# Autodesk Inventor assembly: pinion_assembly
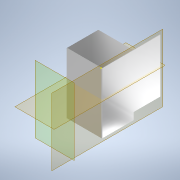
[picture p0: Inventor's stored thumbnail of the model, 180x180]
Saved by Autodesk Inventor 2021 (Build 250183000, 183)
## iProperties
Created: 2021-06-23
Part Number: pinion_assembly
Document SubType Name: Assembly
## Documents named in this file (3)
- C:\Users\ocon0143\OneDrive - Flinders\Advn Mech Design Shared\6_Development\2_Design\inventor\rack_pinion\pinion_assembly.iam
- C:\Users\ocon0143\OneDrive - Flinders\Advn Mech Design Shared\6_Development\2_Design\inventor\support\reel\motor.ipt
- C:\Users\ocon0143\OneDrive - Flinders\Advn Mech Design Shared\6_Development\2_Design\inventor\rack_pinion\rp_box.ipt
## Components (2 placed, 2 different names)
1. motor:1 — Mate:1, Mate:2, Mate:3
2. rp_box:1 — Mate:1, Mate:2, Mate:3
## Relationships (3: Mate 3)
- Mate:1: motor:1 ↔ rp_box:1
- Mate:2: motor:1 ↔ rp_box:1
- Mate:3: motor:1 ↔ rp_box:1
